# Autodesk Inventor assembly: base mg996r 3mm left foot
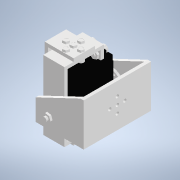
[picture p0: Inventor's stored thumbnail of the model, 180x180]
Saved by Autodesk Inventor 2021.4 (Build 254397000, 397)
## iProperties
Created: 2022-07-09
Part Number: base mg996r 3mm left foot
Document SubType Name: Assembly
Designer: isamu
Author: isamu
## Documents named in this file (5)
- D:\personal_projects\robot\inventor\2021\base mg996r 3mm left foot.iam
- D:\personal_projects\robot\inventor\2021\base mg996r 3mm frame bottom.iam
- D:\personal_projects\robot\exports\frames\servo frame mg996 foot.ipt
- D:\personal_projects\robot\exports\screws\m2 nuts.ipt
- D:\personal_projects\robot\exports\screws\m4 nuts.ipt
## Components (7 placed, 4 different names)
1. base mg996r 3mm frame bottom:1 [sub-assembly] — Mate:1, Mate:2, Mate:3
2. servo frame mg996 foot:1 — Insert:1, Insert:2, Insert:3, Insert:4, Insert:5, Mate:1, Mate:2, Mate:3
3. m2 nuts:1 — Insert:1
4. m2 nuts:2 — Insert:2
5. m2 nuts:3 — Insert:3
6. m2 nuts:4 — Insert:4
7. m4 nuts:1 — Insert:5
## Relationships (8: Insert 5, Mate 3)
- Insert:1: servo frame mg996 foot:1 ↔ m2 nuts:1
- Insert:2: servo frame mg996 foot:1 ↔ m2 nuts:2
- Insert:3: servo frame mg996 foot:1 ↔ m2 nuts:3
- Insert:4: servo frame mg996 foot:1 ↔ m2 nuts:4
- Insert:5: servo frame mg996 foot:1 ↔ m4 nuts:1
- Mate:1: base mg996r 3mm frame bottom:1 ↔ servo frame mg996 foot:1
- Mate:2: base mg996r 3mm frame bottom:1 ↔ servo frame mg996 foot:1
- Mate:3: base mg996r 3mm frame bottom:1 ↔ servo frame mg996 foot:1
